# Autodesk Inventor assembly: 222_onering_soro
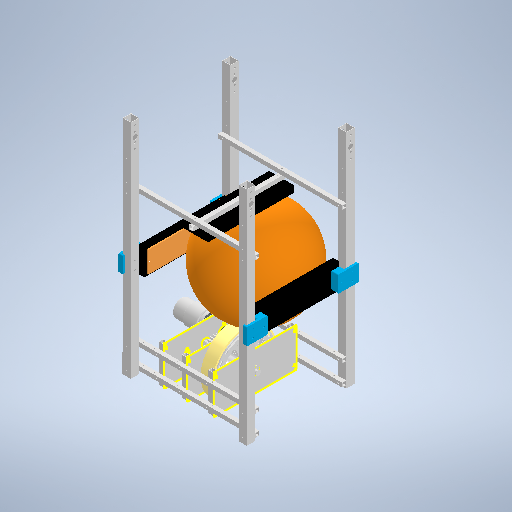
[picture p0: Inventor's stored thumbnail of the model, 512x512]
Saved by Autodesk Inventor 2025.1 (Build 291241000, 241)
## iProperties
Created: 2024-10-08
Part Number: 222_onering_soro
Document SubType Name: Assembly
Designer: yuki0520
Author: yuki0520
## Documents named in this file (8)
- C:\Users\yuki0520\OneDrive\ドキュメント\Inventor\2025_nhk\tanaka\nageru\onering\222_onering_soro.iam
- C:\Users\yuki0520\OneDrive\ドキュメント\Inventor\2025_nhk\tanaka\nageru\pakuriz\001_pakutta_L.iam
- C:\Users\yuki0520\OneDrive\ドキュメント\Inventor\2025_nhk\tanaka\nageru\pakuriz\kaku_1010_530.ipt
- C:\Users\yuki0520\OneDrive\ドキュメント\Inventor\2025_nhk\tanaka\object\ball.ipt
- C:\Users\yuki0520\OneDrive\ドキュメント\Inventor\2025_nhk\tanaka\nageru\pakuriz\TH22_soroban_sn.ipt
- C:\Users\yuki0520\OneDrive\ドキュメント\Inventor\2025_nhk\tanaka\nageru\pakuriz\soroban_hold.ipt
- C:\Users\yuki0520\OneDrive\ドキュメント\Inventor\2025_nhk\tanaka\nageru\onering\kaku_1010_300.ipt
- C:\Users\yuki0520\OneDrive\ドキュメント\Inventor\2025_nhk\tanaka\nageru\onering\kaku_1010_230.ipt
## Components (16 placed, 7 different names)
1. 001_pakutta_L:1 [sub-assembly] — 挿入:9, 正接:1, 挿入:24, 挿入:25, 挿入:28, 挿入:29, 挿入:30, 挿入:31, 挿入:32
2. kaku_1010_530:1 — 挿入:9, 挿入:17, 挿入:18, 挿入:30, 挿入:43
3. kaku_1010_530:2 — 挿入:28, 挿入:29, 挿入:41, 挿入:48, 挿入:49
4. ball:1 — 正接:1, 正接:3, 正接:4
5. kaku_1010_530:3 — 挿入:24, 挿入:25, 挿入:26, 挿入:27, 挿入:40
6. TH22_soroban_sn:1 — 挿入:23, 挿入:35
7. TH22_soroban_sn:2 — 挿入:19, 挿入:20, 正接:3
8. soroban_hold:1 — 挿入:17, 挿入:18, 挿入:20
9. soroban_hold:2 — 挿入:19, 挿入:48, 挿入:49
10. soroban_hold:3 — 挿入:23, 挿入:26, 挿入:27
11. TH22_soroban_sn:3 — 挿入:46, 挿入:47, 正接:4
12. kaku_1010_530:4 — 挿入:31, 挿入:32, 挿入:33, 挿入:34, 挿入:42
13. soroban_hold:4 — 挿入:33, 挿入:34, 挿入:35
14. kaku_1010_300:1 — 挿入:42, 挿入:43, 挿入:45
15. kaku_1010_300:2 — 挿入:40, 挿入:41, 挿入:44
16. kaku_1010_230:1 — 挿入:44, 挿入:45, 挿入:46, 挿入:47
## Relationships (31: Insert 28, Tangent 3)
- 挿入:9 [Insert]: 001_pakutta_L:1 ↔ kaku_1010_530:1
- 正接:1 [Tangent]: 001_pakutta_L:1 ↔ ball:1
- 挿入:17 [Insert]: kaku_1010_530:1 ↔ soroban_hold:1
- 挿入:18 [Insert]: kaku_1010_530:1 ↔ soroban_hold:1
- 挿入:19 [Insert]: TH22_soroban_sn:2 ↔ soroban_hold:2
- 挿入:20 [Insert]: TH22_soroban_sn:2 ↔ soroban_hold:1
- 挿入:23 [Insert]: TH22_soroban_sn:1 ↔ soroban_hold:3
- 正接:3 [Tangent]: ball:1 ↔ TH22_soroban_sn:2
- 挿入:24 [Insert]: 001_pakutta_L:1 ↔ kaku_1010_530:3
- 挿入:25 [Insert]: 001_pakutta_L:1 ↔ kaku_1010_530:3
- 挿入:26 [Insert]: kaku_1010_530:3 ↔ soroban_hold:3
- 挿入:27 [Insert]: kaku_1010_530:3 ↔ soroban_hold:3
- 挿入:28 [Insert]: 001_pakutta_L:1 ↔ kaku_1010_530:2
- 挿入:29 [Insert]: 001_pakutta_L:1 ↔ kaku_1010_530:2
- 挿入:30 [Insert]: 001_pakutta_L:1 ↔ kaku_1010_530:1
- 挿入:31 [Insert]: 001_pakutta_L:1 ↔ kaku_1010_530:4
- 挿入:32 [Insert]: 001_pakutta_L:1 ↔ kaku_1010_530:4
- 挿入:33 [Insert]: kaku_1010_530:4 ↔ soroban_hold:4
- 挿入:34 [Insert]: kaku_1010_530:4 ↔ soroban_hold:4
- 挿入:35 [Insert]: TH22_soroban_sn:1 ↔ soroban_hold:4
- 挿入:40 [Insert]: kaku_1010_530:3 ↔ kaku_1010_300:2
- 挿入:41 [Insert]: kaku_1010_530:2 ↔ kaku_1010_300:2
- 挿入:42 [Insert]: kaku_1010_530:4 ↔ kaku_1010_300:1
- 挿入:43 [Insert]: kaku_1010_530:1 ↔ kaku_1010_300:1
- 挿入:44 [Insert]: kaku_1010_300:2 ↔ kaku_1010_230:1
- 挿入:45 [Insert]: kaku_1010_300:1 ↔ kaku_1010_230:1
- 挿入:46 [Insert]: TH22_soroban_sn:3 ↔ kaku_1010_230:1
- 挿入:47 [Insert]: TH22_soroban_sn:3 ↔ kaku_1010_230:1
- 挿入:48 [Insert]: kaku_1010_530:2 ↔ soroban_hold:2
- 挿入:49 [Insert]: kaku_1010_530:2 ↔ soroban_hold:2
- 正接:4 [Tangent]: ball:1 ↔ TH22_soroban_sn:3
